# Autodesk Inventor assembly: still pipe
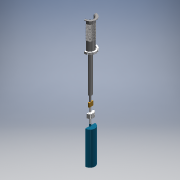
[picture p0: Inventor's stored thumbnail of the model, 180x180]
Saved by Autodesk Inventor 2018 (Build 220112000, 112)
## iProperties
Created: 2019-01-14
Part Number: still pipe
Document SubType Name: Assembly
Designer: Admin
Author: Admin
## Documents named in this file (9)
- C:\Users\Admin\Documents\Cryostat\CAD\still pipe.iam
- C:\Users\Admin\Documents\Cryostat\CAD\KF50 bellows.ipt
- C:\Users\Admin\Documents\Cryostat\CAD\universal connector.ipt
- C:\Users\Admin\Documents\Cryostat\CAD\1in ss pipe.ipt
- C:\Users\Admin\Documents\Cryostat\CAD\adapter.ipt
- C:\Users\Admin\Documents\Cryostat\CAD\heatsink.ipt
- C:\Users\Admin\Documents\Cryostat\CAD\brassbushing2.ipt
- C:\Users\Admin\Documents\Cryostat\CAD\minifridge.ipt
- C:\Users\Admin\Documents\Cryostat\CAD\universal connector male.ipt
## Components (8 placed, 8 different names)
1. KF50 bellows:1 — Mate:16, Flush:2
2. universal connector:1 — Mate:24, Mate:26, Mate:27, Mate:28
3. 1in ss pipe:3 — Mate:15, Flush:1, Mate:17, Mate:31, Mate:32
4. adapter:1 — Mate:15, Flush:1, Mate:16, Flush:2, Mate:19, Mate:34, Mate:35
5. heatsink:1 — Mate:17, Mate:19, Mate:34, Mate:35
6. brassbushing2:1 — Mate:24, Mate:31, Mate:32
7. minifridge:1 — Mate:29, Mate:30
8. universal connector male:1 — Mate:26, Mate:27, Mate:28, Mate:29, Mate:30
## Relationships (16: Mate 14, Flush 2)
- Mate:15: 1in ss pipe:3 ↔ adapter:1
- Flush:1: 1in ss pipe:3 ↔ adapter:1
- Mate:16: KF50 bellows:1 ↔ adapter:1
- Flush:2: KF50 bellows:1 ↔ adapter:1
- Mate:17: 1in ss pipe:3 ↔ heatsink:1
- Mate:19: adapter:1 ↔ heatsink:1
- Mate:24: universal connector:1 ↔ brassbushing2:1
- Mate:26: universal connector:1 ↔ universal connector male:1
- Mate:27: universal connector:1 ↔ universal connector male:1
- Mate:28: universal connector:1 ↔ universal connector male:1
- Mate:29: minifridge:1 ↔ universal connector male:1
- Mate:30: minifridge:1 ↔ universal connector male:1
- Mate:31: 1in ss pipe:3 ↔ brassbushing2:1
- Mate:32: 1in ss pipe:3 ↔ brassbushing2:1
- Mate:34: adapter:1 ↔ heatsink:1
- Mate:35: adapter:1 ↔ heatsink:1
